# Autodesk Inventor assembly: main
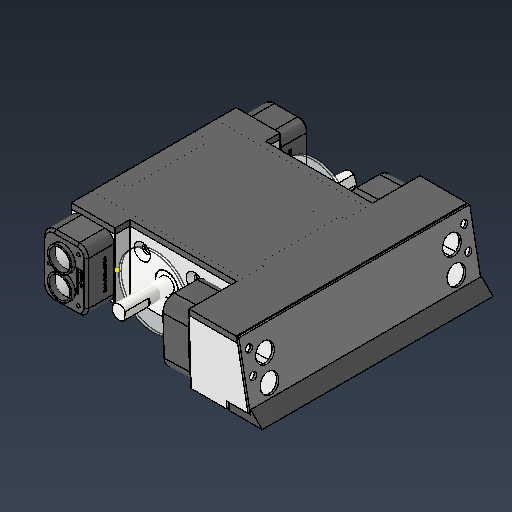
[picture p0: Inventor's stored thumbnail of the model, 512x512]
Saved by Autodesk Inventor 2026.2 (Build 302298010, 298A)
## iProperties
Created: 2026-03-09
Part Number: main
Document SubType Name: Assembly
Designer: szymo
Mass: 382.308 g
Surface Area: 1101.17 cm^2
Volume: 160.883 cm^3
Density: 2.37631 g/cm^3
Author: szymo
## Documents named in this file (22)
- D:\tech\robotyka\robots\evangelion-turbo\inventor-project\main.iam
- D:\tech\robotyka\robots\evangelion-turbo\inventor-project\drive-train.iam
- D:\tech\robotyka\robots\evangelion-turbo\inventor-project\LUNA.ipt
- D:\tech\robotyka\robots\evangelion-turbo\inventor-project\3s450mah.ipt
- D:\tech\robotyka\robots\evangelion-turbo\inventor-project\KTIR-Board.ipt
- D:\tech\robotyka\robots\evangelion-turbo\inventor-project\Left_gearbox.ipt
- D:\tech\robotyka\robots\evangelion-turbo\inventor-project\BearigHoldLeft.ipt
- D:\tech\robotyka\robots\evangelion-turbo\inventor-project\Right_gearbox.ipt
- D:\tech\robotyka\robots\evangelion-turbo\inventor-project\BearigHoldRight.ipt
- D:\tech\robotyka\robots\evangelion-turbo\inventor-project\LeftGearboxCover.ipt
- D:\tech\robotyka\robots\evangelion-turbo\inventor-project\plug.ipt
- D:\tech\robotyka\robots\evangelion-turbo\inventor-project\FonrtMount.ipt
- D:\tech\robotyka\robots\evangelion-turbo\inventor-project\RightGearboxCover.ipt
- D:\tech\robotyka\robots\evangelion-turbo\inventor-project\PCB_interface.ipt
- D:\tech\robotyka\robots\evangelion-turbo\inventor-project\TypC_port\TypC_port\TypC_port.ipt
- D:\tech\robotyka\robots\evangelion-turbo\inventor-project\0.96 oled\0.96 oled\0.96 oled.ipt
- D:\tech\robotyka\robots\evangelion-turbo\inventor-project\THMU 13 (SMD JOYSTICK)\THMU 13 (SMD JOYSTICK)\THMU 13 (SMD JOYSTICK).ipt
- D:\tech\robotyka\robots\evangelion-turbo\inventor-project\PCB_Motors.ipt
- D:\tech\robotyka\robots\evangelion-turbo\inventor-project\PCB_Controller.ipt
- D:\tech\robotyka\robots\evangelion-turbo\inventor-project\PCB_Holder_Floor.ipt
- D:\tech\robotyka\robots\evangelion-turbo\inventor-project\SteelFront.ipt
- D:\tech\robotyka\robots\evangelion-turbo\inventor-project\Ceiling.ipt
## Components (27 placed, 21 different names)
1. drive-train:1 [sub-assembly] — Flush:2, Flush:3, Flush:4, Mate:2, Mate:3, Tangent:1, Mate:9, Angle:3, Mate:13, Mate:15, Mate:16, Tangent:2, Flush:61, Mate:18
2. 3s450mah:1 — Flush:8, Tangent:1, Flush:9
3. Ceiling:1 — Flush:64
4. LUNA:2 — Mate:1, Mate:3, Angle:2, Mate:11, Flush:48, Flush:49, Flush:50
5. LUNA:1 — Flush:5, Mate:2, Angle:1, Mate:12
6. LUNA:3 — Flush:22, Flush:23, Mate:6
7. LUNA:4 — Flush:24, Flush:25, Mate:7
8. KTIR-Board:1 — Flush:10, Flush:11, Flush:13
9. KTIR-Board:2 — Mate:4, Flush:12, Flush:14
10. KTIR-Board:4 — Flush:17, Flush:27, Mate:6, Mate:18
11. KTIR-Board:5 — Flush:28, Flush:29, Mate:7, Mate:19
12. Left_gearbox:1 — Flush:33, Flush:37
13. BearigHoldLeft:1 — Flush:37, Flush:38, Mate:16
14. LeftGearboxCover:1 — Flush:43, Mate:13, Flush:46
15. Right_gearbox:1 — Flush:40, Flush:61, Flush:63
16. BearigHoldRight:1 — Flush:42, Mate:15
17. RightGearboxCover:1 — Flush:52
18. SteelFront:1 — Flush:62
19. plug:1 — Mate:10, Flush:45, Mate:20
20. FonrtMount:1 — Flush:47, Flush:48, Flush:49, Flush:50
21. PCB_Holder_Floor:1 — Flush:60
22. PCB_Motors:1 — Flush:55, Flush:57, Tangent:2, Mate:17
23. PCB_Controller:1 — Flush:58, Flush:59, Mate:17
24. PCB_interface:1 — Mate:14, Flush:55, Flush:57, Flush:58, Flush:59
25. TypC_port:1
26. THMU 13 (SMD JOYSTICK):1
27. 0.96 oled:1 — Mate:14
## Relationships (71: Flush 48, Mate 18, Angle 3, Tangent 2)
- Flush:2 (0.65 mm): drive-train:1
- Flush:3 (-17.65 mm): drive-train:1
- Flush:4 (0.65 mm): drive-train:1
- Flush:5 (49.5 mm): LUNA:1
- Mate:1 (-49.5 mm): LUNA:2
- Mate:2 (18.732 mm): drive-train:1 ↔ LUNA:1
- Mate:3 (18.732 mm): drive-train:1 ↔ LUNA:2
- Angle:1 (-2 deg): LUNA:1
- Angle:2 (182 deg): LUNA:2
- Flush:8 (6.5 mm): 3s450mah:1
- Tangent:1 (0.65 mm): drive-train:1 ↔ 3s450mah:1
- Flush:9 (-31.5 mm): 3s450mah:1
- Flush:10 (-49 mm): KTIR-Board:1
- Mate:4 (-49 mm): KTIR-Board:2
- Flush:11 (0.13 mm): KTIR-Board:1
- Flush:12 (0.13 mm): KTIR-Board:2
- Flush:13 (66.232 mm): KTIR-Board:1
- Flush:14 (-66.232 mm): KTIR-Board:2
- Flush:17: KTIR-Board:4
- Flush:22: LUNA:3
- Flush:23 (1 mm): LUNA:3
- Flush:24 (1 mm): LUNA:4
- Flush:25: LUNA:4
- Flush:27 (0.5 mm): KTIR-Board:4
- Flush:28 (0.5 mm): KTIR-Board:5
- Flush:29: KTIR-Board:5
- Mate:6: LUNA:3 ↔ KTIR-Board:4
- Mate:7: LUNA:4 ↔ KTIR-Board:5
- Flush:32 (-19.75 mm)
- Flush:33: Left_gearbox:1
- Flush:34 (-23 mm)
- Flush:36 (-17.65 mm)
- Flush:37: Left_gearbox:1 ↔ BearigHoldLeft:1
- Flush:38: BearigHoldLeft:1
- Flush:39 (19.75 mm)
- Flush:40: Right_gearbox:1
- Flush:41 (17.65 mm)
- Flush:42: BearigHoldRight:1
- Mate:9: drive-train:1
- Angle:3 (0 deg): drive-train:1
- Flush:43 (1.8 mm): LeftGearboxCover:1
- Mate:10: plug:1
- Flush:45: plug:1
- Mate:11: LUNA:2
- Mate:12: LUNA:1
- Mate:13: drive-train:1 ↔ LeftGearboxCover:1
- Flush:46: LeftGearboxCover:1
- Flush:47: FonrtMount:1
- Flush:48: LUNA:2 ↔ FonrtMount:1
- Flush:49: LUNA:2 ↔ FonrtMount:1
- Flush:50: LUNA:2 ↔ FonrtMount:1
- Flush:51 (26.95 mm)
- Flush:52: RightGearboxCover:1
- Flush:53 (-29 mm)
- Mate:14: PCB_interface:1 ↔ 0.96 oled:1
- Flush:55: PCB_Motors:1 ↔ PCB_interface:1
- Flush:57 (0.1 mm): PCB_Motors:1 ↔ PCB_interface:1
- Mate:15: drive-train:1 ↔ BearigHoldRight:1
- Mate:16: drive-train:1 ↔ BearigHoldLeft:1
- Tangent:2 (5 mm): drive-train:1 ↔ PCB_Motors:1
- Flush:58: PCB_Controller:1 ↔ PCB_interface:1
- Flush:59 (0.1 mm): PCB_Controller:1 ↔ PCB_interface:1
- Mate:17 (3 mm): PCB_Motors:1 ↔ PCB_Controller:1
- Flush:60: PCB_Holder_Floor:1
- Flush:61: drive-train:1 ↔ Right_gearbox:1
- Mate:18 (0.5 mm): drive-train:1 ↔ KTIR-Board:4
- Mate:19 (20.25 mm): KTIR-Board:5
- Flush:62: SteelFront:1
- Flush:63: Right_gearbox:1
- Flush:64: Ceiling:1
- Mate:20 (-97 mm): plug:1
